# Autodesk Inventor assembly: ГЛАЗ НОВЫЙ СБОРКА
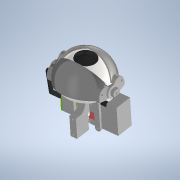
[picture p0: Inventor's stored thumbnail of the model, 180x180]
Saved by Autodesk Inventor 2020 (Build 240168000, 168)
## iProperties
Created: 2022-02-16
Part Number: ГЛАЗ НОВЫЙ СБОРКА
Document SubType Name: Assembly
Designer: Администратор
Author: Администратор
## Documents named in this file (14)
- C:\Users\glazovaes\Downloads\ГЛАЗ НОВЫЙ СБОРКА.iam
- C:\Users\glazovaes\Downloads\верхнее веко.ipt
- C:\Users\glazovaes\Downloads\держалка глаза.ipt
- C:\Users\glazovaes\Downloads\шатун движенияглаза.ipt
- C:\Users\glazovaes\Downloads\связующий сервы движения глаз.ipt
- C:\Users\glazovaes\Downloads\связующий сервы век.ipt
- C:\Users\glazovaes\Downloads\нижний шатун век.ipt
- C:\Users\glazovaes\Downloads\нижнее веко.ipt
- C:\Users\glazovaes\Downloads\держалка сервы движения глаз.ipt
- C:\Users\glazovaes\Downloads\держалка сервы век.ipt
- C:\Users\glazovaes\Downloads\SERVO.ipt
- C:\Users\glazovaes\Downloads\верхний шатун века_ЗЕРКАЛО.ipt
- C:\Users\glazovaes\Downloads\зрачок_ЗЕРКАЛО.ipt
- C:\Users\glazovaes\Downloads\белок глаза_ЗЕРКАЛО.ipt
## Components (14 placed, 13 different names)
1. шатун движенияглаза:1 — Совмещение:28, Совмещение:29, Совмещение:30, Совмещение:31
2. связующий сервы движения глаз:1 — Совмещение:16, Совмещение:17, Совмещение:20
3. связующий сервы век:1 — Совмещение:30, Совмещение:31, Совмещение:38
4. верхнее веко — Совмещение:5, Совмещение:6, Совмещение:7, Совмещение:8, Совмещение:9, Совмещение:11, Совмещение:12
5. держалка сервы движения глаз:1 — Совмещение:32, Совмещение:33, Совмещение:34, Совмещение:35, Совмещение:36, Совмещение:37
6. держалка сервы век:1 — Совмещение:21, Совмещение:22, Совмещение:23
7. держалка глаза:1 — Совмещение:5, Совмещение:6, Совмещение:7, Совмещение:10, Совмещение:18, Совмещение:19, Угол:1, Совмещение:26, Совмещение:27, Совмещение:32, Совмещение:33, Совмещение:34
8. нижнее веко — Совмещение:8, Совмещение:9, Совмещение:10, Совмещение:13, Совмещение:14
9. SERVO:1 — Совмещение:18, Совмещение:19, Угол:1, Совмещение:20, Совмещение:21, Совмещение:22, Совмещение:23
10. SERVO:2 — Совмещение:35, Совмещение:36, Совмещение:37, Совмещение:38
11. нижний шатун век:1 — Совмещение:13, Совмещение:14, Совмещение:15, Совмещение:16
12. верхний шатун века_ЗЕРКАЛО:1 — Совмещение:11, Совмещение:12, Совмещение:15, Совмещение:17
13. зрачок_ЗЕРКАЛО:1 — Совмещение:24, Совмещение:25
14. белок глаза_ЗЕРКАЛО:1 — Совмещение:24, Совмещение:25, Совмещение:26, Совмещение:27, Совмещение:28, Совмещение:29
## Relationships (35: Mate 34, Angle 1)
- Совмещение:5 [Mate]: верхнее веко ↔ держалка глаза:1
- Совмещение:6 [Mate]: верхнее веко ↔ держалка глаза:1
- Совмещение:7 [Mate]: верхнее веко ↔ держалка глаза:1
- Совмещение:8 [Mate]: верхнее веко ↔ нижнее веко
- Совмещение:9 [Mate]: верхнее веко ↔ нижнее веко
- Совмещение:10 [Mate]: держалка глаза:1 ↔ нижнее веко
- Совмещение:11 [Mate]: верхнее веко ↔ верхний шатун века_ЗЕРКАЛО:1
- Совмещение:12 [Mate]: верхнее веко ↔ верхний шатун века_ЗЕРКАЛО:1
- Совмещение:13 [Mate]: нижнее веко ↔ нижний шатун век:1
- Совмещение:14 [Mate]: нижнее веко ↔ нижний шатун век:1
- Совмещение:15 [Mate]: нижний шатун век:1 ↔ верхний шатун века_ЗЕРКАЛО:1
- Совмещение:16 [Mate]: связующий сервы движения глаз:1 ↔ нижний шатун век:1
- Совмещение:17 [Mate]: связующий сервы движения глаз:1 ↔ верхний шатун века_ЗЕРКАЛО:1
- Совмещение:18 [Mate]: держалка глаза:1 ↔ SERVO:1
- Совмещение:19 [Mate]: держалка глаза:1 ↔ SERVO:1
- Угол:1 [Angle] (0 deg): держалка глаза:1 ↔ SERVO:1
- Совмещение:20 [Mate]: связующий сервы движения глаз:1 ↔ SERVO:1
- Совмещение:21 [Mate]: держалка сервы век:1 ↔ SERVO:1
- Совмещение:22 [Mate]: держалка сервы век:1 ↔ SERVO:1
- Совмещение:23 [Mate]: держалка сервы век:1 ↔ SERVO:1
- Совмещение:24 [Mate]: зрачок_ЗЕРКАЛО:1 ↔ белок глаза_ЗЕРКАЛО:1
- Совмещение:25 [Mate]: зрачок_ЗЕРКАЛО:1 ↔ белок глаза_ЗЕРКАЛО:1
- Совмещение:26 [Mate]: держалка глаза:1 ↔ белок глаза_ЗЕРКАЛО:1
- Совмещение:27 [Mate]: держалка глаза:1 ↔ белок глаза_ЗЕРКАЛО:1
- Совмещение:28 [Mate]: шатун движенияглаза:1 ↔ белок глаза_ЗЕРКАЛО:1
- Совмещение:29 [Mate]: шатун движенияглаза:1 ↔ белок глаза_ЗЕРКАЛО:1
- Совмещение:30 [Mate]: шатун движенияглаза:1 ↔ связующий сервы век:1
- Совмещение:31 [Mate]: шатун движенияглаза:1 ↔ связующий сервы век:1
- Совмещение:32 [Mate]: держалка сервы движения глаз:1 ↔ держалка глаза:1
- Совмещение:33 [Mate]: держалка сервы движения глаз:1 ↔ держалка глаза:1
- Совмещение:34 [Mate]: держалка сервы движения глаз:1 ↔ держалка глаза:1
- Совмещение:35 [Mate]: держалка сервы движения глаз:1 ↔ SERVO:2
- Совмещение:36 [Mate]: держалка сервы движения глаз:1 ↔ SERVO:2
- Совмещение:37 [Mate]: держалка сервы движения глаз:1 ↔ SERVO:2
- Совмещение:38 [Mate]: связующий сервы век:1 ↔ SERVO:2
